(part 1 of 2)
# Autodesk Inventor assembly: gasienica_zlozenie
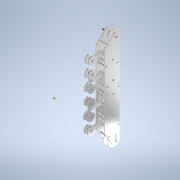
[picture p0: Inventor's stored thumbnail of the model, 180x180]
Saved by Autodesk Inventor 2020.3 (Build 243373000, 373)
## iProperties
Created: 2021-10-24
Part Number: gasienica_zlozenie
Document SubType Name: Assembly
Designer: patry
Author: patry
## Documents named in this file (41)
- C:\Users\patry\Desktop\Semestr 7\Inzynierka\Projekt inventor\Ariadna_inzynierka\Workspaces\Obszar roboczy\Obszar roboczy\Naped\Zawieszenie_v3\gasienica_zlozenie.iam
- C:\Users\patry\Desktop\Semestr 7\Inzynierka\Projekt inventor\Ariadna_inzynierka\Workspaces\Obszar roboczy\Obszar roboczy\Naped\Zawieszenie_v3\plyta_glowna_V3.ipt
- C:\Users\patry\Desktop\Semestr 7\Inzynierka\Projekt inventor\Ariadna_inzynierka\Workspaces\Obszar roboczy\Obszar roboczy\Naped\Sruby\M6_nut_5mm_MIR1.ipt
- C:\Users\patry\Desktop\Semestr 7\Inzynierka\Projekt inventor\Ariadna_inzynierka\Workspaces\Obszar roboczy\Obszar roboczy\Naped\Sruby\M6x65_MIR1.ipt
- C:\Users\patry\Desktop\Semestr 7\Inzynierka\Projekt inventor\Ariadna_inzynierka\Workspaces\Obszar roboczy\Obszar roboczy\Naped\Kola\kolo_przednie.iam
- C:\Users\patry\Desktop\Semestr 7\Inzynierka\Projekt inventor\Ariadna_inzynierka\Workspaces\Obszar roboczy\Obszar roboczy\Naped\Sruby\M5x65.ipt
- C:\Users\patry\Desktop\Semestr 7\Inzynierka\Projekt inventor\Ariadna_inzynierka\Workspaces\Obszar roboczy\Obszar roboczy\Naped\Sruby\M5_nut_5mm.ipt
- C:\Users\patry\Desktop\Semestr 7\Inzynierka\Projekt inventor\Ariadna_inzynierka\Workspaces\Obszar roboczy\Obszar roboczy\Naped\Sruby\dystans_miedzy_plytami.ipt
- C:\Users\patry\Desktop\Semestr 7\Inzynierka\Projekt inventor\Ariadna_inzynierka\Workspaces\Obszar roboczy\Obszar roboczy\Naped\Zawieszenie_v3\glowny_wahacz.ipt
- C:\Users\patry\Desktop\Semestr 7\Inzynierka\Projekt inventor\Ariadna_inzynierka\Workspaces\Obszar roboczy\Obszar roboczy\Naped\Zawieszenie_v3\ramie_1_wahacza.ipt
- C:\Users\patry\Desktop\Semestr 7\Inzynierka\Projekt inventor\Ariadna_inzynierka\Workspaces\Obszar roboczy\Obszar roboczy\Naped\Zawieszenie_v3\ramie_2_wahacza.ipt
- C:\Users\patry\Desktop\Semestr 7\Inzynierka\Projekt inventor\Ariadna_inzynierka\Workspaces\Obszar roboczy\Obszar roboczy\Naped\Zawieszenie_v3\tuleja_TUF106040.ipt
- C:\Users\patry\Desktop\Semestr 7\Inzynierka\Projekt inventor\Ariadna_inzynierka\Workspaces\Obszar roboczy\Obszar roboczy\Naped\Zawieszenie_v3\komplet_kol_V4.iam
- C:\Users\patry\Desktop\Semestr 7\Inzynierka\Projekt inventor\Ariadna_inzynierka\Workspaces\Obszar roboczy\Obszar roboczy\Naped\Sruby\M6_nut_5mm.ipt
- C:\Users\patry\Desktop\Semestr 7\Inzynierka\Projekt inventor\Ariadna_inzynierka\Workspaces\Obszar roboczy\Obszar roboczy\Naped\Zawieszenie_v3\independent_wheel_pair.iam
- C:\Users\patry\Desktop\Semestr 7\Inzynierka\Projekt inventor\Ariadna_inzynierka\Workspaces\Obszar roboczy\Obszar roboczy\Naped\Amortyzator\Korpus.ipt
- C:\Users\patry\Desktop\Semestr 7\Inzynierka\Projekt inventor\Ariadna_inzynierka\Workspaces\Obszar roboczy\Obszar roboczy\Naped\Amortyzator\Tlok.ipt
- C:\Users\patry\Desktop\Semestr 7\Inzynierka\Projekt inventor\Ariadna_inzynierka\Workspaces\Obszar roboczy\Obszar roboczy\Naped\Amortyzator\Nakretka.ipt
- C:\Users\patry\Desktop\Semestr 7\Inzynierka\Projekt inventor\Ariadna_inzynierka\Workspaces\Obszar roboczy\Obszar roboczy\Naped\Zawieszenie_v3\glowny_wahacz_zewn.ipt
- C:\Users\patry\Desktop\Semestr 7\Inzynierka\Projekt inventor\Ariadna_inzynierka\Workspaces\Obszar roboczy\Obszar roboczy\Naped\Sruby\M8_nut_6.5mm_MIR1.ipt
- C:\Users\patry\Desktop\Semestr 7\Inzynierka\Projekt inventor\Ariadna_inzynierka\Workspaces\Obszar roboczy\Obszar roboczy\Naped\Sruby\M8x80_threaded_MIR1.ipt
- C:\Users\patry\Desktop\Semestr 7\Inzynierka\Projekt inventor\Ariadna_inzynierka\Workspaces\Obszar roboczy\Obszar roboczy\Naped\Sruby\M8_pad_MIR1.ipt
- C:\Users\patry\Desktop\Semestr 7\Inzynierka\Projekt inventor\Ariadna_inzynierka\Workspaces\Obszar roboczy\Obszar roboczy\Naped\Lozyska\608ZZ-8mm\bearings-608zz-80018-1.snapshot.1\608zz_MIR1.ipt
- C:\Users\patry\Desktop\Semestr 7\Inzynierka\Projekt inventor\Ariadna_inzynierka\Workspaces\Obszar roboczy\Obszar roboczy\Naped\Kola\kolo_napedowe.iam
- C:\Users\patry\Desktop\Semestr 7\Inzynierka\Projekt inventor\Ariadna_inzynierka\Workspaces\Obszar roboczy\Obszar roboczy\Naped\Sruby\M6_25_shaft.ipt
- C:\Users\patry\Desktop\Semestr 7\Inzynierka\Projekt inventor\Ariadna_inzynierka\Workspaces\Obszar roboczy\Obszar roboczy\Naped\Sruby\M5_70_shaft.ipt
- C:\Users\patry\Desktop\Semestr 7\Inzynierka\Projekt inventor\Ariadna_inzynierka\Workspaces\Obszar roboczy\Obszar roboczy\Naped\Sruby\M3_16_shaft.ipt
- C:\Users\patry\Desktop\Semestr 7\Inzynierka\Projekt inventor\Ariadna_inzynierka\Workspaces\Obszar roboczy\Obszar roboczy\Naped\Sruby\M3_nut_2,5mm.ipt
- C:\Users\patry\Desktop\Semestr 7\Inzynierka\Projekt inventor\Ariadna_inzynierka\Workspaces\Obszar roboczy\Obszar roboczy\Naped\Zawieszenie_v3\wspornik_amortyzatora.ipt
- C:\Users\patry\Desktop\Semestr 7\Inzynierka\Projekt inventor\Ariadna_inzynierka\Workspaces\Obszar roboczy\Obszar roboczy\Naped\Sruby\M6_40_shaft.ipt
- C:\Users\patry\Desktop\Semestr 7\Inzynierka\Projekt inventor\Ariadna_inzynierka\Workspaces\Obszar roboczy\Obszar roboczy\Naped\Sruby\tuleja_M6_M10_7.ipt
- C:\Users\patry\Desktop\Semestr 7\Inzynierka\Projekt inventor\Ariadna_inzynierka\Workspaces\Obszar roboczy\Obszar roboczy\Naped\Sruby\M6_1,25_pad.ipt
- C:\Users\patry\Desktop\Semestr 7\Inzynierka\Projekt inventor\Ariadna_inzynierka\Workspaces\Obszar roboczy\Obszar roboczy\Naped\Sruby\M6_70_shaft.ipt
- C:\Users\patry\Desktop\Semestr 7\Inzynierka\Projekt inventor\Ariadna_inzynierka\Workspaces\Obszar roboczy\Obszar roboczy\Naped\Sruby\M5_40_shaft.ipt
- M5_shaft.ipt
- C:\Users\patry\Desktop\Semestr 7\Inzynierka\Projekt inventor\Ariadna_inzynierka\Workspaces\Obszar roboczy\Obszar roboczy\Naped\Sruby\tuleja_M5_M9_20.ipt
- C:\Users\patry\Desktop\Semestr 7\Inzynierka\Projekt inventor\Ariadna_inzynierka\Workspaces\Obszar roboczy\Obszar roboczy\Naped\Sruby\tuleja_M5_M9_25.ipt
- C:\Users\patry\Desktop\Semestr 7\Inzynierka\Projekt inventor\Ariadna_inzynierka\Workspaces\Obszar roboczy\Obszar roboczy\Naped\Sruby\tuleja_M5_M9_4,5.ipt
- C:\Users\patry\Desktop\Semestr 7\Inzynierka\Projekt inventor\Ariadna_inzynierka\Workspaces\Obszar roboczy\Obszar roboczy\Naped\Kola\holder_wheel_pair.iam
- C:\Users\patry\Desktop\Semestr 7\Inzynierka\Projekt inventor\Ariadna_inzynierka\Workspaces\Obszar roboczy\Obszar roboczy\Naped\Sruby\tuleja_M6_M10_8,5.ipt
- C:\Users\patry\Desktop\Semestr 7\Inzynierka\Projekt inventor\Ariadna_inzynierka\Workspaces\Obszar roboczy\Obszar roboczy\Naped\Sruby\tuleja_M6_M10_13,5.ipt
## Components (293 placed, 39 different names)
1. plyta_glowna_V3:1 — Zestawiające:1, Zestawiające:2, Zestawiające:3, Zestawiające:878, Zestawiające:879, Zestawiające:880
2. plyta_glowna_V3:2 — Zestawiające:1, Zestawiające:2, Zestawiające:3, Zestawiające:11, Zestawiające:12, Zestawiające:19, Zestawiające:20, Zestawiające:21, Zestawiające:22, Zestawiające:26, Zestawiające:27, Zestawiające:354, Równoległe:15, Zestawiające:615, Zestawiające:616, Zestawiające:617, Zestawiające:618, Zestawiające:747, Zestawiające:748, Zestawiające:749, Zestawiające:750, Zestawiające:877, Zestawiające:1006, Zestawiające:1009, Zestawiające:1011, Zestawiające:1012
3. M6_nut_5mm_MIR1:1
4. M6x65_MIR1:1 — Zestawiające:11, Zestawiające:12
5. M6_nut_5mm_MIR1:2
6. M6_nut_5mm_MIR1:3
7. kolo_przednie:1 [sub-assembly]
8. M5x65:1 — Zestawiające:14, Zestawiające:15, Zestawiające:19, Zestawiające:20
9. M5_nut_5mm:1
10. dystans_miedzy_plytami:1 — Zestawiające:14, Zestawiające:15
11. M5x65:2 — Zestawiające:21, Zestawiające:22
12. M5_nut_5mm:2
13. dystans_miedzy_plytami:2
14. M5x65:3 — Zestawiające:26, Zestawiające:27
15. M5_nut_5mm:3
16. dystans_miedzy_plytami:3
17. M8_nut_6.5mm_MIR1:1
18. M8x80_threaded_MIR1:1
19. M8_nut_6.5mm_MIR1:2
20. M8_nut_6.5mm_MIR1:3
21. M8_pad_MIR1:1
22. M8_pad_MIR1:2
23. M8_pad_MIR1:3
24. M8_pad_MIR1:4
25. 608zz_MIR1:1
26. 608zz_MIR1:2 — Zestawiające:354, Równoległe:15
27. kolo_napedowe:1 [sub-assembly]
28. glowny_wahacz:3
29. ramie_1_wahacza:3
30. ramie_2_wahacza:3
31. tuleja_TUF106040:9
32. tuleja_TUF106040:10
33. tuleja_TUF106040:11
34. tuleja_TUF106040:12
35. komplet_kol_V4:2 [sub-assembly]
36. glowny_wahacz:4
37. tuleja_TUF106040:13
38. tuleja_TUF106040:14
39. ramie_2_wahacza:4
40. tuleja_TUF106040:15
41. tuleja_TUF106040:16
42. M6_nut_5mm:11
43. M6_nut_5mm:12
44. Korpus:2
45. Tlok:2
46. Nakretka:2
47. M5_nut_5mm:10
48. M6_25_shaft:2
49. M6_nut_5mm:13
50. M5_70_shaft:2 — Zestawiające:618
51. ramie_1_wahacza:4
52. M5_nut_5mm:11
53. M3_16_shaft:2
54. M3_nut_2,5mm:3
55. M3_nut_2,5mm:4
56. wspornik_amortyzatora:3
57. wspornik_amortyzatora:4
58. M6_40_shaft:3
59. M6_40_shaft:4
60. M6_nut_5mm:14
61. M6_nut_5mm:15
62. M6_nut_5mm:16
63. tuleja_M6_M10_7:3
64. tuleja_M6_M10_7:4
65. M6_1,25_pad:9
66. M6_1,25_pad:10
67. M6_1,25_pad:11
68. M6_1,25_pad:12
69. M6_1,25_pad:13
70. M6_1,25_pad:14
71. M6_1,25_pad:15
72. M6_1,25_pad:16
73. M6_70_shaft:3 — Zestawiające:616
74. M6_70_shaft:4 — Zestawiające:615
75. M6_nut_5mm:17
76. M6_nut_5mm:18 — Zestawiające:617
77. M6_nut_5mm:19
78. M6_nut_5mm:20
79. M5_shaft:3
80. M5_shaft:4
81. M5_nut_5mm:12
82. M5_nut_5mm:13
83. M5_nut_5mm:14
84. M5_nut_5mm:15
85. tuleja_M5_M9_20:2
86. tuleja_M5_M9_25:2
87. tuleja_M5_M9_4,5:5
88. tuleja_M5_M9_4,5:6
89. tuleja_M5_M9_4,5:7
90. tuleja_M5_M9_4,5:8
91. holder_wheel_pair:2 [sub-assembly]
92. tuleja_M6_M10_8,5:3
93. tuleja_M6_M10_13,5:3
94. tuleja_M6_M10_8,5:4
95. tuleja_M6_M10_13,5:4
96. glowny_wahacz:5
97. ramie_1_wahacza:5
98. ramie_2_wahacza:5
99. tuleja_TUF106040:17
100. tuleja_TUF106040:18
101. tuleja_TUF106040:19
102. tuleja_TUF106040:20
103. komplet_kol_V4:3 [sub-assembly]
104. glowny_wahacz:6
105. tuleja_TUF106040:21
106. tuleja_TUF106040:22
107. ramie_2_wahacza:6
108. tuleja_TUF106040:23
109. tuleja_TUF106040:24
110. M6_nut_5mm:21
111. M6_nut_5mm:22
112. Korpus:3
113. Tlok:3
114. Nakretka:3
115. M5_nut_5mm:16
116. M6_25_shaft:3
117. M6_nut_5mm:23
118. M5_70_shaft:3
119. ramie_1_wahacza:6
120. M5_nut_5mm:17
121. M3_16_shaft:3
122. M3_nut_2,5mm:5
123. M3_nut_2,5mm:6
124. wspornik_amortyzatora:5
125. wspornik_amortyzatora:6
126. M6_40_shaft:5
127. M6_40_shaft:6
128. M6_nut_5mm:24
129. M6_nut_5mm:25
130. M6_nut_5mm:26
131. tuleja_M6_M10_7:5
132. tuleja_M6_M10_7:6
133. M6_1,25_pad:17
134. M6_1,25_pad:18
135. M6_1,25_pad:19
136. M6_1,25_pad:20
137. M6_1,25_pad:21
138. M6_1,25_pad:22
139. M6_1,25_pad:23
140. M6_1,25_pad:24
141. M6_70_shaft:5
142. M6_70_shaft:6 — Zestawiające:748
143. M6_nut_5mm:27
144. M6_nut_5mm:28
145. M6_nut_5mm:29
146. M6_nut_5mm:30
147. M5_shaft:5
148. M5_shaft:6
149. M5_nut_5mm:18
150. M5_nut_5mm:19
151. M5_nut_5mm:20
152. M5_nut_5mm:21
153. tuleja_M5_M9_20:3
154. tuleja_M5_M9_25:3 — Zestawiające:750
155. tuleja_M5_M9_4,5:9
156. tuleja_M5_M9_4,5:10
157. tuleja_M5_M9_4,5:11
158. tuleja_M5_M9_4,5:12
159. holder_wheel_pair:3 [sub-assembly]
160. tuleja_M6_M10_8,5:5
161. tuleja_M6_M10_13,5:5 — Zestawiające:747, Zestawiające:749
162. tuleja_M6_M10_8,5:6
163. tuleja_M6_M10_13,5:6
164. ramie_1_wahacza:7
165. ramie_2_wahacza:7
166. tuleja_TUF106040:25
167. tuleja_TUF106040:26
168. tuleja_TUF106040:27
169. tuleja_TUF106040:28
170. tuleja_TUF106040:29
171. tuleja_TUF106040:30
172. ramie_2_wahacza:8
173. tuleja_TUF106040:31
174. tuleja_TUF106040:32
175. M6_nut_5mm:32
176. Korpus:4
177. Tlok:4
178. Nakretka:4
179. M5_nut_5mm:22
180. M5_70_shaft:4
181. ramie_1_wahacza:8
182. M5_nut_5mm:23
183. M3_16_shaft:4
184. M3_nut_2,5mm:7
185. M3_nut_2,5mm:8
186. wspornik_amortyzatora:7
187. wspornik_amortyzatora:8
188. M6_40_shaft:7
189. M6_40_shaft:8
190. M6_nut_5mm:34
191. M6_nut_5mm:35
192. M6_nut_5mm:36
193. tuleja_M6_M10_7:7
194. tuleja_M6_M10_7:8
195. M6_1,25_pad:25
196. M6_1,25_pad:26
197. M6_1,25_pad:27
198. M6_1,25_pad:28
199. M6_1,25_pad:29
200. M6_1,25_pad:30
201. M6_1,25_pad:31
202. M6_1,25_pad:32
203. M6_70_shaft:7 — Zestawiające:879
204. M6_70_shaft:8 — Zestawiające:878
205. M6_nut_5mm:37
206. M6_nut_5mm:38
207. M6_nut_5mm:39
208. M6_nut_5mm:40
209. M5_shaft:7
210. M5_shaft:8
211. M5_nut_5mm:24
212. M5_nut_5mm:25
213. M5_nut_5mm:26
214. M5_nut_5mm:27
215. tuleja_M5_M9_20:4
216. tuleja_M5_M9_25:4 — Zestawiające:880
217. tuleja_M5_M9_4,5:13
218. tuleja_M5_M9_4,5:14
219. tuleja_M5_M9_4,5:15
220. tuleja_M5_M9_4,5:16
221. glowny_wahacz_zewn:1 — Zestawiające:881, Zestawiające:882, Zestawiające:884
222. glowny_wahacz_zewn:2
223. tuleja_M6_M10_8,5:7
224. tuleja_M6_M10_13,5:7 — Zestawiające:877
225. tuleja_M6_M10_13,5:8
226. tuleja_M6_M10_8,5:8
227. independent_wheel_pair:1 [sub-assembly] — Zestawiające:881, Zestawiające:882, Zestawiające:883
228. tuleja_M6_M10_7:9 — Zestawiające:883, Zestawiające:884
229. ramie_1_wahacza:9
230. ramie_2_wahacza:9
231. tuleja_TUF106040:33
232. tuleja_TUF106040:34
233. tuleja_TUF106040:35
234. tuleja_TUF106040:36
235. tuleja_TUF106040:37 — Zestawiające:1010
236. tuleja_TUF106040:38
237. ramie_2_wahacza:10
238. tuleja_TUF106040:39
239. tuleja_TUF106040:40
240. M6_nut_5mm:41
241. Korpus:5
242. Tlok:5
243. Nakretka:5
244. M5_nut_5mm:28 — Zestawiające:1006
245. M5_70_shaft:5
246. ramie_1_wahacza:10
247. M5_nut_5mm:29
248. M3_16_shaft:5
249. M3_nut_2,5mm:9
250. M3_nut_2,5mm:10
251. wspornik_amortyzatora:9
252. wspornik_amortyzatora:10
253. M6_40_shaft:9
254. M6_40_shaft:10
255. M6_nut_5mm:42
256. M6_nut_5mm:43
257. M6_nut_5mm:44
258. tuleja_M6_M10_7:10
259. tuleja_M6_M10_7:11
260. M6_1,25_pad:33
261. M6_1,25_pad:34
262. M6_1,25_pad:35
263. M6_1,25_pad:36
264. M6_1,25_pad:37
265. M6_1,25_pad:38
266. M6_1,25_pad:39
267. M6_1,25_pad:40
268. M6_70_shaft:9
269. M6_70_shaft:10 — Zestawiające:1009, Zestawiające:1010
270. M6_nut_5mm:45
271. M6_nut_5mm:46
272. M6_nut_5mm:47
273. M6_nut_5mm:48
274. M5_shaft:9
275. M5_shaft:10
276. M5_nut_5mm:30
277. M5_nut_5mm:31
278. M5_nut_5mm:32
279. M5_nut_5mm:33
280. tuleja_M5_M9_20:5
281. tuleja_M5_M9_25:5 — Zestawiające:1012
282. tuleja_M5_M9_4,5:17
283. tuleja_M5_M9_4,5:18
284. tuleja_M5_M9_4,5:19
285. tuleja_M5_M9_4,5:20
286. glowny_wahacz_zewn:3 — Zestawiające:1007, Zestawiające:1008
287. glowny_wahacz_zewn:4
288. tuleja_M6_M10_8,5:9
289. tuleja_M6_M10_13,5:9 — Zestawiające:1011
290. tuleja_M6_M10_13,5:10
291. tuleja_M6_M10_8,5:10
292. independent_wheel_pair:2 [sub-assembly] — Zestawiające:1007
293. tuleja_M6_M10_7:12 — Zestawiające:1008
## Relationships (630: Mate 565, Flush 45, Angle 16, CylindricalJoint 4)
- Zestawiające:1 [Mate]: plyta_glowna_V3:1 ↔ plyta_glowna_V3:2
- Zestawiające:2 [Mate]: plyta_glowna_V3:1 ↔ plyta_glowna_V3:2
- Zestawiające:3 [Mate] (50 mm): plyta_glowna_V3:1 ↔ plyta_glowna_V3:2
- [Flush]: M6_nut_5mm_MIR1:1 ↔ M6x65_MIR1:1
- [Mate]: M6_nut_5mm_MIR1:1 ↔ M6x65_MIR1:1
- [Mate] (12 mm): M6_nut_5mm_MIR1:1 ↔ M6_nut_5mm_MIR1:2
- [Mate]: M6x65_MIR1:1 ↔ M6_nut_5mm_MIR1:2
- [Mate] (12 mm): M6x65_MIR1:1 ↔ M6_nut_5mm_MIR1:3
- [Mate]: M6x65_MIR1:1 ↔ M6_nut_5mm_MIR1:3
- [Mate]: M6x65_MIR1:1 ↔ kolo_przednie:1
- [Mate]: M6_nut_5mm_MIR1:3 ↔ kolo_przednie:1
- Zestawiające:11 [Mate]: plyta_glowna_V3:2 ↔ M6x65_MIR1:1
- Zestawiające:12 [Mate]: plyta_glowna_V3:2 ↔ M6x65_MIR1:1
- [Mate]: M5x65:1 ↔ M5_nut_5mm:1
- [Flush]: M5x65:1 ↔ M5_nut_5mm:1
- Zestawiające:14 [Mate]: M5x65:1 ↔ dystans_miedzy_plytami:1
- Zestawiające:15 [Mate] (5 mm): M5x65:1 ↔ dystans_miedzy_plytami:1
- [Mate]: M5x65:2 ↔ M5_nut_5mm:2
- [Flush]: M5x65:2 ↔ M5_nut_5mm:2
- [Mate]: M5x65:2 ↔ dystans_miedzy_plytami:2
- [Mate] (5 mm): M5x65:2 ↔ dystans_miedzy_plytami:2
- Zestawiające:19 [Mate]: plyta_glowna_V3:2 ↔ M5x65:1
- Zestawiające:20 [Mate]: plyta_glowna_V3:2 ↔ M5x65:1
- Zestawiające:21 [Mate]: plyta_glowna_V3:2 ↔ M5x65:2
- Zestawiające:22 [Mate]: plyta_glowna_V3:2 ↔ M5x65:2
- [Mate]: M5x65:3 ↔ M5_nut_5mm:3
- [Flush]: M5x65:3 ↔ M5_nut_5mm:3
- [Mate]: M5x65:3 ↔ dystans_miedzy_plytami:3
- [Mate] (5 mm): M5x65:3 ↔ dystans_miedzy_plytami:3
- Zestawiające:26 [Mate]: plyta_glowna_V3:2 ↔ M5x65:3
- Zestawiające:27 [Mate]: plyta_glowna_V3:2 ↔ M5x65:3
- [Mate]: M8_nut_6.5mm_MIR1:1 ↔ M8x80_threaded_MIR1:1
- [Mate]: M8x80_threaded_MIR1:1 ↔ M8_nut_6.5mm_MIR1:2
- [Mate]: M8x80_threaded_MIR1:1 ↔ M8_nut_6.5mm_MIR1:3
- [Mate]: M8_nut_6.5mm_MIR1:1 ↔ M8_pad_MIR1:1
- [Mate] (7 mm): M8x80_threaded_MIR1:1 ↔ M8_pad_MIR1:1
- [Mate]: M8x80_threaded_MIR1:1 ↔ M8_pad_MIR1:1
- [Mate]: M8_nut_6.5mm_MIR1:1 ↔ M8_pad_MIR1:2
- [Mate]: M8x80_threaded_MIR1:1 ↔ M8_pad_MIR1:2
- [Mate] (7 mm): M8_nut_6.5mm_MIR1:2 ↔ M8_pad_MIR1:3
- [Mate]: M8_nut_6.5mm_MIR1:3 ↔ M8_pad_MIR1:3
- [Mate]: M8x80_threaded_MIR1:1 ↔ M8_pad_MIR1:3
- [Mate]: M8_nut_6.5mm_MIR1:3 ↔ M8_pad_MIR1:4
- [Mate] (31 mm): M8_pad_MIR1:2 ↔ M8_pad_MIR1:4
- [Mate]: M8x80_threaded_MIR1:1 ↔ M8_pad_MIR1:4
- [Mate]: M8x80_threaded_MIR1:1 ↔ 608zz_MIR1:1
- [Mate]: M8_nut_6.5mm_MIR1:2 ↔ 608zz_MIR1:1
- [Mate]: M8x80_threaded_MIR1:1 ↔ 608zz_MIR1:2
- [Mate]: M8x80_threaded_MIR1:1 ↔ 608zz_MIR1:2
- [Mate]: M8x80_threaded_MIR1:1 ↔ kolo_napedowe:1
- [Mate]: M8_pad_MIR1:2 ↔ kolo_napedowe:1
- Zestawiające:354 [Mate]: plyta_glowna_V3:2 ↔ 608zz_MIR1:2
- Równoległe:15 [Flush] (1 mm): plyta_glowna_V3:2 ↔ 608zz_MIR1:2
- [Mate]: ramie_2_wahacza:3 ↔ tuleja_TUF106040:9
- [Mate]: ramie_2_wahacza:3 ↔ tuleja_TUF106040:9
- [Angle] (0 deg): ramie_2_wahacza:3 ↔ tuleja_TUF106040:9
- [Mate]: ramie_1_wahacza:3 ↔ tuleja_TUF106040:12
- [Mate]: ramie_1_wahacza:3 ↔ tuleja_TUF106040:12
- [Angle] (0 deg): ramie_1_wahacza:3 ↔ tuleja_TUF106040:12
- [Mate]: glowny_wahacz:3 ↔ komplet_kol_V4:2
- [Mate]: komplet_kol_V4:2 ↔ glowny_wahacz:4
- [Mate]: komplet_kol_V4:2 ↔ glowny_wahacz:4
- [Mate]: glowny_wahacz:3 ↔ komplet_kol_V4:2
- [Mate] (2.5 mm): glowny_wahacz:3 ↔ tuleja_TUF106040:9
- [Mate]: ramie_2_wahacza:4 ↔ tuleja_TUF106040:15
- [Mate]: ramie_2_wahacza:4 ↔ tuleja_TUF106040:15
- [Angle] (0 deg): ramie_2_wahacza:4 ↔ tuleja_TUF106040:15
- [Mate] (2.5 mm): glowny_wahacz:4 ↔ tuleja_TUF106040:15
- [Mate]: glowny_wahacz:3 ↔ M6_nut_5mm:11
- [Mate]: Korpus:2 ↔ Tlok:2
- [Angle] (0 deg): Korpus:2 ↔ Tlok:2
- [Mate]: Korpus:2 ↔ Nakretka:2
- [Mate] (5 mm): Korpus:2 ↔ Nakretka:2
- [CylindricalJoint]: Korpus:2 ↔ Tlok:2
- [Mate]: glowny_wahacz:3 ↔ glowny_wahacz:4
- [Mate]: glowny_wahacz:4 ↔ M6_25_shaft:2
- [Flush] (6 mm): glowny_wahacz:4 ↔ M6_25_shaft:2
- [Mate]: M6_25_shaft:2 ↔ M6_nut_5mm:13
- [Mate]: glowny_wahacz:4 ↔ M6_nut_5mm:13
- [Mate]: Korpus:2 ↔ M5_70_shaft:2
- [Flush] (-30 mm): Korpus:2 ↔ M5_70_shaft:2
- [Mate]: M5_nut_5mm:10 ↔ M5_70_shaft:2
- [Mate]: M5_70_shaft:2 ↔ M5_nut_5mm:11
- [Mate] (60 mm): M5_nut_5mm:10 ↔ M5_nut_5mm:11
- [Mate] (30 mm): Korpus:2 ↔ M5_nut_5mm:10
- [Mate]: tuleja_TUF106040:14 ↔ ramie_1_wahacza:4
- [Mate]: tuleja_TUF106040:14 ↔ ramie_1_wahacza:4
- [Mate]: glowny_wahacz:4 ↔ tuleja_TUF106040:15
- [Mate]: tuleja_TUF106040:9 ↔ tuleja_TUF106040:15
- [Mate]: wspornik_amortyzatora:3 ↔ wspornik_amortyzatora:4
- [Mate]: wspornik_amortyzatora:3 ↔ wspornik_amortyzatora:4
- [Mate] (5 mm): wspornik_amortyzatora:3 ↔ wspornik_amortyzatora:4
- [Mate]: M3_16_shaft:2 ↔ wspornik_amortyzatora:4
- [Flush] (-2.5 mm): M3_16_shaft:2 ↔ wspornik_amortyzatora:3
- [Mate]: M3_16_shaft:2 ↔ M3_nut_2,5mm:3
- [Mate]: M3_nut_2,5mm:3 ↔ wspornik_amortyzatora:3
- [Mate]: M3_16_shaft:2 ↔ M3_nut_2,5mm:4
- [Mate]: M3_nut_2,5mm:4 ↔ wspornik_amortyzatora:4
- [Mate]: Tlok:2 ↔ M3_16_shaft:2
- [Mate]: Tlok:2 ↔ wspornik_amortyzatora:4
- [Mate]: tuleja_TUF106040:12 ↔ glowny_wahacz:4
- [Mate] (2.5 mm): tuleja_TUF106040:12 ↔ glowny_wahacz:4
- [Mate] (2.5 mm): glowny_wahacz:3 ↔ tuleja_TUF106040:14
- [Mate]: glowny_wahacz:3 ↔ tuleja_TUF106040:14
- [Mate]: ramie_1_wahacza:3 ↔ wspornik_amortyzatora:3
- [Mate]: ramie_1_wahacza:3 ↔ wspornik_amortyzatora:3
- [Mate] (4.5 mm): ramie_1_wahacza:3 ↔ wspornik_amortyzatora:3
- [Mate]: tuleja_TUF106040:12 ↔ M6_40_shaft:3
- [Flush] (7 mm): ramie_1_wahacza:3 ↔ M6_40_shaft:3
- [Mate]: tuleja_TUF106040:15 ↔ M6_40_shaft:4
- [Flush] (7 mm): ramie_2_wahacza:4 ↔ M6_40_shaft:4
- [Mate]: M6_nut_5mm:12 ↔ M6_40_shaft:3
- [Mate]: ramie_1_wahacza:3 ↔ M6_nut_5mm:12
- [Mate]: M6_40_shaft:3 ↔ M6_nut_5mm:14
- [Mate]: ramie_1_wahacza:4 ↔ M6_nut_5mm:14
- [Mate]: M6_40_shaft:4 ↔ M6_nut_5mm:15
- [Mate]: ramie_2_wahacza:3 ↔ M6_nut_5mm:15
- [Mate]: M6_40_shaft:4 ↔ M6_nut_5mm:16
- [Mate]: ramie_2_wahacza:4 ↔ M6_nut_5mm:16
- [Mate]: M6_40_shaft:3 ↔ tuleja_M6_M10_7:3
- [Mate]: glowny_wahacz:3 ↔ tuleja_M6_M10_7:3
- [Mate]: M6_40_shaft:4 ↔ tuleja_M6_M10_7:4
- [Mate]: glowny_wahacz:4 ↔ tuleja_M6_M10_7:4
- [Mate]: M6_1,25_pad:9 ↔ M6_1,25_pad:10
- [Mate]: M6_1,25_pad:9 ↔ M6_1,25_pad:10
- [Mate]: M6_40_shaft:3 ↔ M6_1,25_pad:9
- [Mate]: glowny_wahacz:3 ↔ M6_1,25_pad:9
- [Mate]: M6_1,25_pad:11 ↔ M6_1,25_pad:12
- [Mate]: M6_1,25_pad:11 ↔ M6_1,25_pad:12
- [Mate]: M6_40_shaft:3 ↔ M6_1,25_pad:11
- [Mate]: tuleja_TUF106040:12 ↔ M6_1,25_pad:11
- [Mate]: M6_1,25_pad:13 ↔ M6_1,25_pad:14
- [Mate]: M6_1,25_pad:13 ↔ M6_1,25_pad:14
- [Mate]: M6_40_shaft:4 ↔ M6_1,25_pad:13
- [Mate]: glowny_wahacz:3 ↔ M6_1,25_pad:13
- [Mate]: M6_1,25_pad:15 ↔ M6_1,25_pad:16
- [Mate]: M6_1,25_pad:15 ↔ M6_1,25_pad:16
- [Mate]: M6_40_shaft:4 ↔ M6_1,25_pad:15
- [Mate]: tuleja_TUF106040:15 ↔ M6_1,25_pad:15
- [Mate]: M5_70_shaft:2 ↔ M6_70_shaft:3
- [Flush]: M5_70_shaft:2 ↔ M6_70_shaft:4
- [Mate]: M6_70_shaft:4 ↔ M6_nut_5mm:17
- [Mate]: M6_70_shaft:4 ↔ M6_nut_5mm:18
- [Mate] (60 mm): M6_nut_5mm:17 ↔ M6_nut_5mm:18
- [Flush]: M5_nut_5mm:10 ↔ M6_nut_5mm:18
- [Mate] (60 mm): M6_nut_5mm:19 ↔ M6_nut_5mm:20
- [Mate]: M6_nut_5mm:19 ↔ M6_nut_5mm:20
- [Mate]: M6_70_shaft:3 ↔ M6_nut_5mm:19
- [Flush]: M5_nut_5mm:10 ↔ M6_nut_5mm:20
- [Mate]: ramie_1_wahacza:3 ↔ M5_shaft:3
- [Flush] (7 mm): ramie_1_wahacza:3 ↔ M5_shaft:3
- [Mate]: ramie_1_wahacza:3 ↔ M5_shaft:4
- [Flush] (7 mm): ramie_1_wahacza:3 ↔ M5_shaft:4
- [Mate]: M5_shaft:4 ↔ M5_nut_5mm:12
- [Mate]: ramie_1_wahacza:3 ↔ M5_nut_5mm:12
- [Mate]: M5_shaft:3 ↔ M5_nut_5mm:13
- [Mate]: ramie_1_wahacza:3 ↔ M5_nut_5mm:13
- [Mate]: M5_shaft:3 ↔ M5_nut_5mm:14
- [Mate]: ramie_1_wahacza:4 ↔ M5_nut_5mm:14
- [Mate]: M5_shaft:4 ↔ M5_nut_5mm:15
- [Mate]: ramie_1_wahacza:4 ↔ M5_nut_5mm:15
- [Mate]: M5_70_shaft:2 ↔ tuleja_M5_M9_20:2
- [Mate]: Korpus:2 ↔ tuleja_M5_M9_20:2
- [Mate]: M5_70_shaft:2 ↔ tuleja_M5_M9_25:2
- [Mate]: Korpus:2 ↔ tuleja_M5_M9_25:2
- [Mate]: M5_shaft:3 ↔ tuleja_M5_M9_4,5:5
- [Mate]: ramie_1_wahacza:4 ↔ tuleja_M5_M9_4,5:5
- [Mate]: M5_shaft:3 ↔ tuleja_M5_M9_4,5:6
- [Mate]: ramie_1_wahacza:3 ↔ tuleja_M5_M9_4,5:6
- [Mate]: M5_shaft:4 ↔ tuleja_M5_M9_4,5:7
- [Mate]: ramie_1_wahacza:4 ↔ tuleja_M5_M9_4,5:7
- [Mate]: M5_shaft:4 ↔ tuleja_M5_M9_4,5:8
- [Mate]: ramie_1_wahacza:3 ↔ tuleja_M5_M9_4,5:8
- [Mate]: glowny_wahacz:4 ↔ holder_wheel_pair:2
- [Flush]: komplet_kol_V4:2 ↔ holder_wheel_pair:2
- [Mate]: tuleja_TUF106040:16 ↔ M6_70_shaft:3
- [Mate]: ramie_2_wahacza:4 ↔ tuleja_TUF106040:16
- [Mate]: ramie_2_wahacza:4 ↔ tuleja_TUF106040:16
- [Mate]: tuleja_TUF106040:10 ↔ M6_70_shaft:3
- [Mate]: ramie_2_wahacza:3 ↔ tuleja_TUF106040:10
- [Mate]: ramie_2_wahacza:3 ↔ tuleja_TUF106040:10
- [Mate]: tuleja_TUF106040:13 ↔ M6_70_shaft:4
- [Mate]: tuleja_TUF106040:13 ↔ ramie_1_wahacza:4
- [Mate]: tuleja_TUF106040:13 ↔ ramie_1_wahacza:4
- [Mate]: tuleja_TUF106040:11 ↔ M6_70_shaft:4
- [Mate]: ramie_1_wahacza:3 ↔ tuleja_TUF106040:11
- [Mate]: ramie_1_wahacza:3 ↔ tuleja_TUF106040:11
- [Mate]: M6_70_shaft:3 ↔ tuleja_M6_M10_8,5:3
- [Mate]: tuleja_TUF106040:16 ↔ tuleja_M6_M10_8,5:3
- [Mate]: M6_70_shaft:3 ↔ tuleja_M6_M10_13,5:3
- [Mate]: tuleja_TUF106040:10 ↔ tuleja_M6_M10_13,5:3
- [Mate]: M6_70_shaft:4 ↔ tuleja_M6_M10_13,5:4
- [Mate]: tuleja_TUF106040:13 ↔ tuleja_M6_M10_13,5:4
- [Mate]: M6_70_shaft:4 ↔ tuleja_M6_M10_8,5:4
- [Mate]: tuleja_TUF106040:11 ↔ tuleja_M6_M10_8,5:4
- [Mate]: M6_nut_5mm:11 ↔ M6_25_shaft:2
- [Mate]: glowny_wahacz:3 ↔ M6_nut_5mm:11
- Zestawiające:615 [Mate]: plyta_glowna_V3:2 ↔ M6_70_shaft:4
- Zestawiające:616 [Mate]: plyta_glowna_V3:2 ↔ M6_70_shaft:3
- Zestawiające:617 [Mate]: plyta_glowna_V3:2 ↔ M6_nut_5mm:18
- Zestawiające:618 [Mate]: plyta_glowna_V3:2 ↔ M5_70_shaft:2
- [Mate]: ramie_2_wahacza:5 ↔ tuleja_TUF106040:17
- [Mate]: ramie_2_wahacza:5 ↔ tuleja_TUF106040:17
- [Angle] (0 deg): ramie_2_wahacza:5 ↔ tuleja_TUF106040:17
- [Mate]: ramie_1_wahacza:5 ↔ tuleja_TUF106040:20
- [Mate]: ramie_1_wahacza:5 ↔ tuleja_TUF106040:20
- [Angle] (0 deg): ramie_1_wahacza:5 ↔ tuleja_TUF106040:20
- [Mate]: glowny_wahacz:5 ↔ komplet_kol_V4:3
- [Mate]: komplet_kol_V4:3 ↔ glowny_wahacz:6
- [Mate]: komplet_kol_V4:3 ↔ glowny_wahacz:6
- [Mate]: glowny_wahacz:5 ↔ komplet_kol_V4:3
- [Mate] (2.5 mm): glowny_wahacz:5 ↔ tuleja_TUF106040:17
- [Mate]: ramie_2_wahacza:6 ↔ tuleja_TUF106040:23
- [Mate]: ramie_2_wahacza:6 ↔ tuleja_TUF106040:23
- [Angle] (0 deg): ramie_2_wahacza:6 ↔ tuleja_TUF106040:23
- [Mate] (2.5 mm): glowny_wahacz:6 ↔ tuleja_TUF106040:23
- [Mate]: glowny_wahacz:5 ↔ M6_nut_5mm:21
- [Mate]: Korpus:3 ↔ Tlok:3
- [Angle] (0 deg): Korpus:3 ↔ Tlok:3
- [Mate]: Korpus:3 ↔ Nakretka:3
- [Mate] (5 mm): Korpus:3 ↔ Nakretka:3
- [CylindricalJoint]: Korpus:3 ↔ Tlok:3
- [Mate]: glowny_wahacz:5 ↔ glowny_wahacz:6
- [Mate]: glowny_wahacz:6 ↔ M6_25_shaft:3
- [Flush] (6 mm): glowny_wahacz:6 ↔ M6_25_shaft:3
- [Mate]: M6_25_shaft:3 ↔ M6_nut_5mm:23
- [Mate]: glowny_wahacz:6 ↔ M6_nut_5mm:23
- [Mate]: Korpus:3 ↔ M5_70_shaft:3
- [Flush] (-30 mm): Korpus:3 ↔ M5_70_shaft:3
- [Mate]: M5_nut_5mm:16 ↔ M5_70_shaft:3
- [Mate]: M5_70_shaft:3 ↔ M5_nut_5mm:17
- [Mate] (60 mm): M5_nut_5mm:16 ↔ M5_nut_5mm:17
- [Mate] (30 mm): Korpus:3 ↔ M5_nut_5mm:16
- [Mate]: tuleja_TUF106040:22 ↔ ramie_1_wahacza:6
- [Mate]: tuleja_TUF106040:22 ↔ ramie_1_wahacza:6
- [Mate]: glowny_wahacz:6 ↔ tuleja_TUF106040:23
- [Mate]: tuleja_TUF106040:17 ↔ tuleja_TUF106040:23
- [Mate]: wspornik_amortyzatora:5 ↔ wspornik_amortyzatora:6
- [Mate]: wspornik_amortyzatora:5 ↔ wspornik_amortyzatora:6
- [Mate] (5 mm): wspornik_amortyzatora:5 ↔ wspornik_amortyzatora:6
- [Mate]: M3_16_shaft:3 ↔ wspornik_amortyzatora:6
- [Flush] (-2.5 mm): M3_16_shaft:3 ↔ wspornik_amortyzatora:5
- [Mate]: M3_16_shaft:3 ↔ M3_nut_2,5mm:5
- [Mate]: M3_nut_2,5mm:5 ↔ wspornik_amortyzatora:5
- [Mate]: M3_16_shaft:3 ↔ M3_nut_2,5mm:6
- [Mate]: M3_nut_2,5mm:6 ↔ wspornik_amortyzatora:6
- [Mate]: Tlok:3 ↔ M3_16_shaft:3
- [Mate]: Tlok:3 ↔ wspornik_amortyzatora:6
- [Mate]: tuleja_TUF106040:20 ↔ glowny_wahacz:6
- [Mate] (2.5 mm): tuleja_TUF106040:20 ↔ glowny_wahacz:6
- [Mate] (2.5 mm): glowny_wahacz:5 ↔ tuleja_TUF106040:22
- [Mate]: glowny_wahacz:5 ↔ tuleja_TUF106040:22
- [Mate]: ramie_1_wahacza:5 ↔ wspornik_amortyzatora:5
- [Mate]: ramie_1_wahacza:5 ↔ wspornik_amortyzatora:5
- [Mate] (4.5 mm): ramie_1_wahacza:5 ↔ wspornik_amortyzatora:5
- [Mate]: tuleja_TUF106040:20 ↔ M6_40_shaft:5
- [Flush] (7 mm): ramie_1_wahacza:5 ↔ M6_40_shaft:5
- [Mate]: tuleja_TUF106040:23 ↔ M6_40_shaft:6
- [Flush] (7 mm): ramie_2_wahacza:6 ↔ M6_40_shaft:6
- [Mate]: M6_nut_5mm:22 ↔ M6_40_shaft:5
- [Mate]: ramie_1_wahacza:5 ↔ M6_nut_5mm:22
- [Mate]: M6_40_shaft:5 ↔ M6_nut_5mm:24
- [Mate]: ramie_1_wahacza:6 ↔ M6_nut_5mm:24
- [Mate]: M6_40_shaft:6 ↔ M6_nut_5mm:25
- [Mate]: ramie_2_wahacza:5 ↔ M6_nut_5mm:25
- [Mate]: M6_40_shaft:6 ↔ M6_nut_5mm:26
- [Mate]: ramie_2_wahacza:6 ↔ M6_nut_5mm:26
- [Mate]: M6_40_shaft:5 ↔ tuleja_M6_M10_7:5
- [Mate]: glowny_wahacz:5 ↔ tuleja_M6_M10_7:5
- [Mate]: M6_40_shaft:6 ↔ tuleja_M6_M10_7:6
- [Mate]: glowny_wahacz:6 ↔ tuleja_M6_M10_7:6
- [Mate]: M6_1,25_pad:17 ↔ M6_1,25_pad:18
- [Mate]: M6_1,25_pad:17 ↔ M6_1,25_pad:18
- [Mate]: M6_40_shaft:5 ↔ M6_1,25_pad:17
- [Mate]: glowny_wahacz:5 ↔ M6_1,25_pad:17
- [Mate]: M6_1,25_pad:19 ↔ M6_1,25_pad:20
- [Mate]: M6_1,25_pad:19 ↔ M6_1,25_pad:20
- [Mate]: M6_40_shaft:5 ↔ M6_1,25_pad:19
- [Mate]: tuleja_TUF106040:20 ↔ M6_1,25_pad:19
- [Mate]: M6_1,25_pad:21 ↔ M6_1,25_pad:22
- [Mate]: M6_1,25_pad:21 ↔ M6_1,25_pad:22
- [Mate]: M6_40_shaft:6 ↔ M6_1,25_pad:21
- [Mate]: glowny_wahacz:5 ↔ M6_1,25_pad:21
- [Mate]: M6_1,25_pad:23 ↔ M6_1,25_pad:24
- [Mate]: M6_1,25_pad:23 ↔ M6_1,25_pad:24
- [Mate]: M6_40_shaft:6 ↔ M6_1,25_pad:23
- [Mate]: tuleja_TUF106040:23 ↔ M6_1,25_pad:23
- [Mate]: M5_70_shaft:3 ↔ M6_70_shaft:5
- [Flush]: M5_70_shaft:3 ↔ M6_70_shaft:6
- [Mate]: M6_70_shaft:6 ↔ M6_nut_5mm:27
- [Mate]: M6_70_shaft:6 ↔ M6_nut_5mm:28
- [Mate] (60 mm): M6_nut_5mm:27 ↔ M6_nut_5mm:28
- [Flush]: M5_nut_5mm:16 ↔ M6_nut_5mm:28
- [Mate] (60 mm): M6_nut_5mm:29 ↔ M6_nut_5mm:30
- [Mate]: M6_nut_5mm:29 ↔ M6_nut_5mm:30
- [Mate]: M6_70_shaft:5 ↔ M6_nut_5mm:29
- [Flush]: M5_nut_5mm:16 ↔ M6_nut_5mm:30
- [Mate]: ramie_1_wahacza:5 ↔ M5_shaft:5
- [Flush] (7 mm): ramie_1_wahacza:5 ↔ M5_shaft:5
- [Mate]: ramie_1_wahacza:5 ↔ M5_shaft:6
- [Flush] (7 mm): ramie_1_wahacza:5 ↔ M5_shaft:6
- [Mate]: M5_shaft:6 ↔ M5_nut_5mm:18
- [Mate]: ramie_1_wahacza:5 ↔ M5_nut_5mm:18
- [Mate]: M5_shaft:5 ↔ M5_nut_5mm:19
- [Mate]: ramie_1_wahacza:5 ↔ M5_nut_5mm:19
- [Mate]: M5_shaft:5 ↔ M5_nut_5mm:20
- [Mate]: ramie_1_wahacza:6 ↔ M5_nut_5mm:20
- [Mate]: M5_shaft:6 ↔ M5_nut_5mm:21
- [Mate]: ramie_1_wahacza:6 ↔ M5_nut_5mm:21
- [Mate]: M5_70_shaft:3 ↔ tuleja_M5_M9_20:3
- [Mate]: Korpus:3 ↔ tuleja_M5_M9_20:3
- [Mate]: M5_70_shaft:3 ↔ tuleja_M5_M9_25:3
- [Mate]: Korpus:3 ↔ tuleja_M5_M9_25:3
- [Mate]: M5_shaft:5 ↔ tuleja_M5_M9_4,5:9
- [Mate]: ramie_1_wahacza:6 ↔ tuleja_M5_M9_4,5:9
- [Mate]: M5_shaft:5 ↔ tuleja_M5_M9_4,5:10
- [Mate]: ramie_1_wahacza:5 ↔ tuleja_M5_M9_4,5:10
- [Mate]: M5_shaft:6 ↔ tuleja_M5_M9_4,5:11
- [Mate]: ramie_1_wahacza:6 ↔ tuleja_M5_M9_4,5:11
- [Mate]: M5_shaft:6 ↔ tuleja_M5_M9_4,5:12
- [Mate]: ramie_1_wahacza:5 ↔ tuleja_M5_M9_4,5:12
- [Mate]: glowny_wahacz:6 ↔ holder_wheel_pair:3
- [Flush]: komplet_kol_V4:3 ↔ holder_wheel_pair:3
- [Mate]: tuleja_TUF106040:24 ↔ M6_70_shaft:5
- [Mate]: ramie_2_wahacza:6 ↔ tuleja_TUF106040:24
- [Mate]: ramie_2_wahacza:6 ↔ tuleja_TUF106040:24
- [Mate]: tuleja_TUF106040:18 ↔ M6_70_shaft:5
- [Mate]: ramie_2_wahacza:5 ↔ tuleja_TUF106040:18
- [Mate]: ramie_2_wahacza:5 ↔ tuleja_TUF106040:18
- [Mate]: tuleja_TUF106040:21 ↔ M6_70_shaft:6
- [Mate]: tuleja_TUF106040:21 ↔ ramie_1_wahacza:6
- [Mate]: tuleja_TUF106040:21 ↔ ramie_1_wahacza:6
- [Mate]: tuleja_TUF106040:19 ↔ M6_70_shaft:6
- [Mate]: ramie_1_wahacza:5 ↔ tuleja_TUF106040:19
- [Mate]: ramie_1_wahacza:5 ↔ tuleja_TUF106040:19
- [Mate]: M6_70_shaft:5 ↔ tuleja_M6_M10_8,5:5
- [Mate]: tuleja_TUF106040:24 ↔ tuleja_M6_M10_8,5:5
- [Mate]: M6_70_shaft:5 ↔ tuleja_M6_M10_13,5:5
- [Mate]: tuleja_TUF106040:18 ↔ tuleja_M6_M10_13,5:5
- [Mate]: M6_70_shaft:6 ↔ tuleja_M6_M10_13,5:6
- [Mate]: tuleja_TUF106040:21 ↔ tuleja_M6_M10_13,5:6
- [Mate]: M6_70_shaft:6 ↔ tuleja_M6_M10_8,5:6
- [Mate]: tuleja_TUF106040:19 ↔ tuleja_M6_M10_8,5:6
- [Mate]: M6_nut_5mm:21 ↔ M6_25_shaft:3
- [Mate]: glowny_wahacz:5 ↔ M6_nut_5mm:21
- Zestawiające:747 [Mate]: plyta_glowna_V3:2 ↔ tuleja_M6_M10_13,5:5
- Zestawiające:748 [Mate]: plyta_glowna_V3:2 ↔ M6_70_shaft:6
- Zestawiające:749 [Mate]: plyta_glowna_V3:2 ↔ tuleja_M6_M10_13,5:5
- Zestawiające:750 [Mate]: plyta_glowna_V3:2 ↔ tuleja_M5_M9_25:3
- [Mate]: ramie_2_wahacza:7 ↔ tuleja_TUF106040:25
- [Mate]: ramie_2_wahacza:7 ↔ tuleja_TUF106040:25
- [Angle] (0 deg): ramie_2_wahacza:7 ↔ tuleja_TUF106040:25
- [Mate]: ramie_1_wahacza:7 ↔ tuleja_TUF106040:28
- [Mate]: ramie_1_wahacza:7 ↔ tuleja_TUF106040:28
- [Angle] (0 deg): ramie_1_wahacza:7 ↔ tuleja_TUF106040:28
- [Mate]: ramie_2_wahacza:8 ↔ tuleja_TUF106040:31
- [Mate]: ramie_2_wahacza:8 ↔ tuleja_TUF106040:31
- [Angle] (0 deg): ramie_2_wahacza:8 ↔ tuleja_TUF106040:31
- [Mate]: Korpus:4 ↔ Tlok:4
- [Angle] (0 deg): Korpus:4 ↔ Tlok:4
- [Mate]: Korpus:4 ↔ Nakretka:4
- [Mate] (5 mm): Korpus:4 ↔ Nakretka:4
- [CylindricalJoint]: Korpus:4 ↔ Tlok:4
- [Mate]: Korpus:4 ↔ M5_70_shaft:4
- [Flush] (-30 mm): Korpus:4 ↔ M5_70_shaft:4
- [Mate]: M5_nut_5mm:22 ↔ M5_70_shaft:4
- [Mate]: M5_70_shaft:4 ↔ M5_nut_5mm:23
- [Mate] (60 mm): M5_nut_5mm:22 ↔ M5_nut_5mm:23
- [Mate] (30 mm): Korpus:4 ↔ M5_nut_5mm:22
- [Mate]: tuleja_TUF106040:30 ↔ ramie_1_wahacza:8
- [Mate]: tuleja_TUF106040:29 ↔ ramie_1_wahacza:8
- [Mate]: tuleja_TUF106040:30 ↔ ramie_1_wahacza:8
- [Mate]: tuleja_TUF106040:25 ↔ tuleja_TUF106040:31
- [Mate]: wspornik_amortyzatora:7 ↔ wspornik_amortyzatora:8
- [Mate]: wspornik_amortyzatora:7 ↔ wspornik_amortyzatora:8
- [Mate] (5 mm): wspornik_amortyzatora:7 ↔ wspornik_amortyzatora:8
- [Mate]: M3_16_shaft:4 ↔ wspornik_amortyzatora:8
- [Flush] (-2.5 mm): M3_16_shaft:4 ↔ wspornik_amortyzatora:7
- [Mate]: M3_16_shaft:4 ↔ M3_nut_2,5mm:7
- [Mate]: M3_nut_2,5mm:7 ↔ wspornik_amortyzatora:7
- [Mate]: M3_16_shaft:4 ↔ M3_nut_2,5mm:8
- [Mate]: M3_nut_2,5mm:8 ↔ wspornik_amortyzatora:8
- [Mate]: Tlok:4 ↔ M3_16_shaft:4
- [Mate]: Tlok:4 ↔ wspornik_amortyzatora:8
- [Mate]: ramie_1_wahacza:7 ↔ wspornik_amortyzatora:7
- [Mate]: ramie_1_wahacza:7 ↔ wspornik_amortyzatora:7
- [Mate] (4.5 mm): ramie_1_wahacza:7 ↔ wspornik_amortyzatora:7
- [Mate]: tuleja_TUF106040:28 ↔ M6_40_shaft:7
- [Flush] (7 mm): ramie_1_wahacza:7 ↔ M6_40_shaft:7
- [Mate]: tuleja_TUF106040:31 ↔ M6_40_shaft:8
- [Flush] (7 mm): ramie_2_wahacza:8 ↔ M6_40_shaft:8
- [Mate]: M6_nut_5mm:32 ↔ M6_40_shaft:7
- [Mate]: ramie_1_wahacza:7 ↔ M6_nut_5mm:32
- [Mate]: M6_40_shaft:7 ↔ M6_nut_5mm:34
- [Mate]: ramie_1_wahacza:8 ↔ M6_nut_5mm:34
- [Mate]: M6_40_shaft:8 ↔ M6_nut_5mm:35
- [Mate]: ramie_2_wahacza:7 ↔ M6_nut_5mm:35
- [Mate]: M6_40_shaft:8 ↔ M6_nut_5mm:36
- [Mate]: ramie_2_wahacza:8 ↔ M6_nut_5mm:36
- [Mate]: M6_40_shaft:7 ↔ tuleja_M6_M10_7:7
- [Mate]: M6_40_shaft:8 ↔ tuleja_M6_M10_7:8
- [Mate]: M6_1,25_pad:25 ↔ M6_1,25_pad:26
- [Mate]: M6_1,25_pad:25 ↔ M6_1,25_pad:26
- [Mate]: M6_40_shaft:7 ↔ M6_1,25_pad:25
- [Mate]: M6_1,25_pad:27 ↔ M6_1,25_pad:28
- [Mate]: M6_1,25_pad:27 ↔ M6_1,25_pad:28
- [Mate]: M6_40_shaft:7 ↔ M6_1,25_pad:27
- [Mate]: tuleja_TUF106040:28 ↔ M6_1,25_pad:27
- [Mate]: M6_1,25_pad:29 ↔ M6_1,25_pad:30
- [Mate]: M6_1,25_pad:29 ↔ M6_1,25_pad:30
- [Mate]: M6_40_shaft:8 ↔ M6_1,25_pad:29
- [Mate]: M6_1,25_pad:31 ↔ M6_1,25_pad:32
- [Mate]: M6_1,25_pad:31 ↔ M6_1,25_pad:32
- [Mate]: M6_40_shaft:8 ↔ M6_1,25_pad:31
- [Mate]: tuleja_TUF106040:31 ↔ M6_1,25_pad:31
- [Mate]: M5_70_shaft:4 ↔ M6_70_shaft:7
- [Flush]: M5_70_shaft:4 ↔ M6_70_shaft:8
- [Mate]: M6_70_shaft:8 ↔ M6_nut_5mm:37
- [Mate]: M6_70_shaft:8 ↔ M6_nut_5mm:38
- [Mate] (60 mm): M6_nut_5mm:37 ↔ M6_nut_5mm:38
- [Flush]: M5_nut_5mm:22 ↔ M6_nut_5mm:38
- [Mate] (60 mm): M6_nut_5mm:39 ↔ M6_nut_5mm:40
- [Mate]: M6_nut_5mm:39 ↔ M6_nut_5mm:40
- [Mate]: M6_70_shaft:7 ↔ M6_nut_5mm:39
- [Flush]: M5_nut_5mm:22 ↔ M6_nut_5mm:40
- [Mate]: ramie_1_wahacza:7 ↔ M5_shaft:7
- [Flush] (7 mm): ramie_1_wahacza:7 ↔ M5_shaft:7
- [Mate]: ramie_1_wahacza:7 ↔ M5_shaft:8
- [Flush] (7 mm): ramie_1_wahacza:7 ↔ M5_shaft:8
- [Mate]: M5_shaft:8 ↔ M5_nut_5mm:24
- [Mate]: ramie_1_wahacza:7 ↔ M5_nut_5mm:24
- [Mate]: M5_shaft:7 ↔ M5_nut_5mm:25
- [Mate]: ramie_1_wahacza:7 ↔ M5_nut_5mm:25
- [Mate]: M5_shaft:7 ↔ M5_nut_5mm:26
- [Mate]: ramie_1_wahacza:8 ↔ M5_nut_5mm:26
- [Mate]: M5_shaft:8 ↔ M5_nut_5mm:27
- [Mate]: ramie_1_wahacza:8 ↔ M5_nut_5mm:27
- [Mate]: M5_70_shaft:4 ↔ tuleja_M5_M9_20:4
- [Mate]: Korpus:4 ↔ tuleja_M5_M9_20:4
- [Mate]: M5_70_shaft:4 ↔ tuleja_M5_M9_25:4
- [Mate]: Korpus:4 ↔ tuleja_M5_M9_25:4
- [Mate]: M5_shaft:7 ↔ tuleja_M5_M9_4,5:13
- [Mate]: ramie_1_wahacza:8 ↔ tuleja_M5_M9_4,5:13
- [Mate]: M5_shaft:7 ↔ tuleja_M5_M9_4,5:14
- [Mate]: ramie_1_wahacza:7 ↔ tuleja_M5_M9_4,5:14
- [Mate]: M5_shaft:8 ↔ tuleja_M5_M9_4,5:15
- [Mate]: ramie_1_wahacza:8 ↔ tuleja_M5_M9_4,5:15
- [Mate]: M5_shaft:8 ↔ tuleja_M5_M9_4,5:16
- [Mate]: ramie_1_wahacza:7 ↔ tuleja_M5_M9_4,5:16
- [Mate]: M6_40_shaft:8 ↔ glowny_wahacz_zewn:1
- [Mate]: tuleja_M6_M10_7:8 ↔ glowny_wahacz_zewn:1
- [Mate]: M6_40_shaft:7 ↔ glowny_wahacz_zewn:1
- [Mate]: M6_40_shaft:8 ↔ glowny_wahacz_zewn:2
- [Mate]: M6_40_shaft:7 ↔ glowny_wahacz_zewn:2
- [Mate]: tuleja_TUF106040:30 ↔ M6_40_shaft:7
- [Mate]: M6_1,25_pad:28 ↔ glowny_wahacz_zewn:2
- [Mate]: M6_1,25_pad:32 ↔ glowny_wahacz_zewn:2
- [Mate]: tuleja_M6_M10_7:7 ↔ glowny_wahacz_zewn:1
- [Mate]: M6_1,25_pad:25 ↔ glowny_wahacz_zewn:1
- [Mate]: tuleja_TUF106040:30 ↔ M6_1,25_pad:26
- [Mate]: M6_1,25_pad:29 ↔ glowny_wahacz_zewn:1
- [Mate]: tuleja_TUF106040:25 ↔ M6_1,25_pad:30
- [Mate]: tuleja_TUF106040:29 ↔ ramie_1_wahacza:8
- [Mate]: tuleja_TUF106040:27 ↔ M6_70_shaft:8
- [Mate]: ramie_1_wahacza:7 ↔ tuleja_TUF106040:27
- [Mate]: ramie_1_wahacza:7 ↔ tuleja_TUF106040:27
- [Mate]: tuleja_TUF106040:26 ↔ M6_70_shaft:7
- [Mate]: ramie_2_wahacza:7 ↔ tuleja_TUF106040:26
- [Mate]: ramie_2_wahacza:7 ↔ tuleja_TUF106040:26
- [Mate]: tuleja_TUF106040:32 ↔ M6_70_shaft:7
- [Mate]: ramie_2_wahacza:8 ↔ tuleja_TUF106040:32
- [Mate]: ramie_2_wahacza:8 ↔ tuleja_TUF106040:32
- [Mate]: M6_70_shaft:7 ↔ tuleja_M6_M10_8,5:7
- [Mate]: tuleja_TUF106040:32 ↔ tuleja_M6_M10_8,5:7
- [Mate]: M6_70_shaft:7 ↔ tuleja_M6_M10_13,5:7
- [Mate]: M6_70_shaft:8 ↔ tuleja_M6_M10_13,5:8
- [Mate]: tuleja_TUF106040:29 ↔ tuleja_M6_M10_13,5:8
- [Mate]: tuleja_TUF106040:26 ↔ tuleja_M6_M10_13,5:7
- [Mate]: M6_70_shaft:8 ↔ tuleja_M6_M10_8,5:8
- [Mate]: tuleja_TUF106040:27 ↔ tuleja_M6_M10_8,5:8
- Zestawiające:877 [Mate]: plyta_glowna_V3:2 ↔ tuleja_M6_M10_13,5:7
- Zestawiające:878 [Mate]: plyta_glowna_V3:1 ↔ M6_70_shaft:8
- Zestawiające:879 [Mate]: plyta_glowna_V3:1 ↔ M6_70_shaft:7
- Zestawiające:880 [Mate]: plyta_glowna_V3:1 ↔ tuleja_M5_M9_25:4
- Zestawiające:881 [Mate]: glowny_wahacz_zewn:1 ↔ independent_wheel_pair:1
- Zestawiające:882 [Mate]: glowny_wahacz_zewn:1 ↔ independent_wheel_pair:1
- Zestawiające:883 [Mate]: independent_wheel_pair:1 ↔ tuleja_M6_M10_7:9
- Zestawiające:884 [Mate]: glowny_wahacz_zewn:1 ↔ tuleja_M6_M10_7:9
- [Mate]: ramie_2_wahacza:9 ↔ tuleja_TUF106040:33
- [Mate]: ramie_2_wahacza:9 ↔ tuleja_TUF106040:33
- [Angle] (0 deg): ramie_2_wahacza:9 ↔ tuleja_TUF106040:33
- [Mate]: ramie_1_wahacza:9 ↔ tuleja_TUF106040:36
- [Mate]: ramie_1_wahacza:9 ↔ tuleja_TUF106040:36
- [Angle] (0 deg): ramie_1_wahacza:9 ↔ tuleja_TUF106040:36
- [Mate]: ramie_2_wahacza:10 ↔ tuleja_TUF106040:39
- [Mate]: ramie_2_wahacza:10 ↔ tuleja_TUF106040:39
- [Angle] (0 deg): ramie_2_wahacza:10 ↔ tuleja_TUF106040:39
- [Mate]: Korpus:5 ↔ Tlok:5
- [Angle] (0 deg): Korpus:5 ↔ Tlok:5